# Autodesk Inventor assembly: propeller
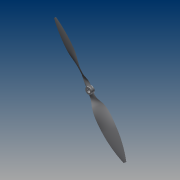
[picture p0: Inventor's stored thumbnail of the model, 180x180]
Saved by Autodesk Inventor 2011 SP1 (Build 150282100, 282)
## iProperties
Created: 2011-07-19
Part Number: propeller
Document SubType Name: Assembly
Designer: Nathan
Author: Nathan
## Documents named in this file (3)
- C:\Users\Nathan\Documents\Inventor\Quadcopter\propeller.iam
- C:\Users\Nathan\Documents\Inventor\Quadcopter\shaft.ipt
- C:\Users\Nathan\Documents\Inventor\Quadcopter\prop.ipt
## Components (3 placed, 2 different names)
1. shaft:1 — Flush:2, Mate:8, Mate:9
2. prop:1 — Mate:7, Flush:1, Flush:2, Mate:9
3. prop:2 — Mate:7, Flush:1, Mate:8
## Relationships (5: Mate 3, Flush 2)
- Mate:7: prop:1 ↔ prop:2
- Flush:1: prop:1 ↔ prop:2
- Flush:2 (3.175 mm): shaft:1 ↔ prop:1
- Mate:8: shaft:1 ↔ prop:2
- Mate:9: shaft:1 ↔ prop:1
